# Autodesk Inventor assembly: upper_arm_004
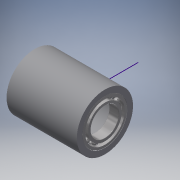
[picture p0: Inventor's stored thumbnail of the model, 180x180]
Saved by Autodesk Inventor 2016 SP1 (Build 200210100, 210)
## iProperties
Created: 2016-06-21
Part Number: upper_arm_004
Document SubType Name: Assembly
Designer: asvsf
Author: asvsf
## Documents named in this file (3)
- C:\Project\Engineering\Suspension\arm_borne.iam
- C:\Project\Engineering\Suspension\Solid1.ipt
- C:\Project\Engineering\Suspension\upper_arm\Design Accelerator\Bearing1.iam
## Components (3 placed, 2 different names)
1. Solid1:1 — Mate:1, Mate:2, Flush:1, Flush:2
2. Bearing:1 [sub-assembly] — Mate:2, Flush:1
3. Bearing:2 [sub-assembly] — Mate:1, Flush:2
## Relationships (4: Mate 2, Flush 2)
- Mate:1: Solid1:1 ↔ Bearing:2
- Mate:2: Solid1:1 ↔ Bearing:1
- Flush:1: Solid1:1 ↔ Bearing:1
- Flush:2: Solid1:1 ↔ Bearing:2
